# Autodesk Inventor assembly: Removedor
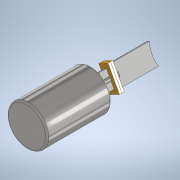
[picture p0: Inventor's stored thumbnail of the model, 180x180]
Saved by Autodesk Inventor 2020.1 (Build 241239000, 239)
## iProperties
Created: 2020-03-26
Part Number: Removedor
Document SubType Name: Assembly
Designer: Daniel
Author: Daniel
## Documents named in this file (4)
- F:\Proyectos\Dog Feeder\Solido\Removedor\Removedor.iam
- F:\Proyectos\Dog Feeder\Solido\Removedor\Acoplador.ipt
- F:\Proyectos\Dog Feeder\Solido\Removedor\Motor DC.ipt
- F:\Proyectos\Dog Feeder\Solido\Removedor\Paleta.ipt
## Components (4 placed, 3 different names)
1. Acoplador:1 — Cylindrical:1, Flush:1, Flush:2, Mate:1
2. Motor DC:1 — Cylindrical:1, Mate:5
3. Paleta:1 — Mate:2, Mate:3, Mate:4, Mate:5
4. Acoplador:2 — Flush:1, Flush:2, Mate:1, Mate:2, Mate:3, Mate:4
## Relationships (8: Mate 5, Flush 2, CylindricalJoint 1)
- Cylindrical:1: Acoplador:1 ↔ Motor DC:1
- Flush:1: Acoplador:1 ↔ Acoplador:2
- Flush:2: Acoplador:1 ↔ Acoplador:2
- Mate:1: Acoplador:1 ↔ Acoplador:2
- Mate:2: Paleta:1 ↔ Acoplador:2
- Mate:3: Paleta:1 ↔ Acoplador:2
- Mate:4: Paleta:1 ↔ Acoplador:2
- Mate:5 (3 mm): Motor DC:1 ↔ Paleta:1
